# Autodesk Inventor assembly: ActiveClimb-ver1-1111-2020
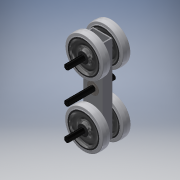
[picture p0: Inventor's stored thumbnail of the model, 180x180]
Saved by Autodesk Inventor 2018 (Build 220112000, 112)
## iProperties
Created: 2020-01-25
Part Number: ActiveClimb-ver1-1111-2020
Document SubType Name: Assembly
Designer: Power Hawks CADD
Author: Power Hawks CADD
## Documents named in this file (5)
- G:\PHRC Design Team\GrabCAD\Power Hawks CAD\2020 Infinite Recharge\Active Climb\Assemblies\ActiveClimb-ver1-1111-2020.iam
- G:\PHRC Design Team\GrabCAD\Power Hawks CAD\2020 Infinite Recharge\Active Climb\Parts\AluminumBar-1111-2020.ipt
- G:\PHRC Design Team\GrabCAD\Power Hawks CAD\Resources\VEXpro Resources\Bearings\0.5inHexFlangedBearing(1.125inx0.313in)-1111-2016.ipt
- G:\PHRC Design Team\GrabCAD\Power Hawks CAD\Resources\VEXpro Resources\Shafts\0.5inThunderHexShaft(5in(4.875))-1111-2016.ipt
- G:\PHRC Design Team\GrabCAD\Power Hawks CAD\Resources\VEXpro Resources\Wheels\4 inch\4inColsonPerformaWheel-1111-2017_MIR.ipt
## Components (14 placed, 4 different names)
1. AluminumBar-1111-2020:1 — Rotational:1, Rotational:2, Rotational:3, Rotational:4, Rotational:5, Rotational:6
2. 0.5inHexFlangedBearing(1.125inx0.313in)-1111-2016:1 — Rotational:1, Insert:7
3. 0.5inHexFlangedBearing(1.125inx0.313in)-1111-2016:2 — Rotational:3, Insert:6
4. 0.5inHexFlangedBearing(1.125inx0.313in)-1111-2016:3 — Rotational:4, Insert:3, Insert:4
5. 0.5inHexFlangedBearing(1.125inx0.313in)-1111-2016:4 — Rotational:2
6. 0.5inHexFlangedBearing(1.125inx0.313in)-1111-2016:5 — Rotational:5, Insert:2
7. 0.5inHexFlangedBearing(1.125inx0.313in)-1111-2016:6 — Rotational:6, Insert:1, Insert:5
8. 0.5inThunderHexShaft(5in(4.875))-1111-2016:1 — Insert:3
9. 0.5inThunderHexShaft(5in(4.875))-1111-2016:2 — Insert:2
10. 0.5inThunderHexShaft(5in(4.875))-1111-2016:3 — Insert:1
11. 4inColsonPerformaWheel-1111-2017_MIR:2 — Insert:4
12. 4inColsonPerformaWheel-1111-2017_MIR:3 — Insert:5
13. 4inColsonPerformaWheel-1111-2017_MIR:4 — Insert:6
14. 4inColsonPerformaWheel-1111-2017_MIR:5 — Insert:7
## Relationships (13: Insert 7, RevoluteJoint 6)
- Rotational:1 [RevoluteJoint]: AluminumBar-1111-2020:1 ↔ 0.5inHexFlangedBearing(1.125inx0.313in)-1111-2016:1
- Rotational:2 [RevoluteJoint]: AluminumBar-1111-2020:1 ↔ 0.5inHexFlangedBearing(1.125inx0.313in)-1111-2016:4
- Rotational:3 [RevoluteJoint]: AluminumBar-1111-2020:1 ↔ 0.5inHexFlangedBearing(1.125inx0.313in)-1111-2016:2
- Rotational:4 [RevoluteJoint]: AluminumBar-1111-2020:1 ↔ 0.5inHexFlangedBearing(1.125inx0.313in)-1111-2016:3
- Rotational:5 [RevoluteJoint]: AluminumBar-1111-2020:1 ↔ 0.5inHexFlangedBearing(1.125inx0.313in)-1111-2016:5
- Rotational:6 [RevoluteJoint]: AluminumBar-1111-2020:1 ↔ 0.5inHexFlangedBearing(1.125inx0.313in)-1111-2016:6
- Insert:1 (-95.25 mm): 0.5inHexFlangedBearing(1.125inx0.313in)-1111-2016:6 ↔ 0.5inThunderHexShaft(5in(4.875))-1111-2016:3
- Insert:2 (-95.25 mm): 0.5inHexFlangedBearing(1.125inx0.313in)-1111-2016:5 ↔ 0.5inThunderHexShaft(5in(4.875))-1111-2016:2
- Insert:3 (-95.25 mm): 0.5inHexFlangedBearing(1.125inx0.313in)-1111-2016:3 ↔ 0.5inThunderHexShaft(5in(4.875))-1111-2016:1
- Insert:4: 0.5inHexFlangedBearing(1.125inx0.313in)-1111-2016:3 ↔ 4inColsonPerformaWheel-1111-2017_MIR:2
- Insert:5: 0.5inHexFlangedBearing(1.125inx0.313in)-1111-2016:6 ↔ 4inColsonPerformaWheel-1111-2017_MIR:3
- Insert:6: 0.5inHexFlangedBearing(1.125inx0.313in)-1111-2016:2 ↔ 4inColsonPerformaWheel-1111-2017_MIR:4
- Insert:7: 0.5inHexFlangedBearing(1.125inx0.313in)-1111-2016:1 ↔ 4inColsonPerformaWheel-1111-2017_MIR:5
